# Autodesk Inventor assembly: Assembly1
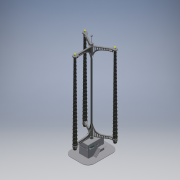
[picture p0: Inventor's stored thumbnail of the model, 180x180]
Saved by Autodesk Inventor 2018 (Build 220112000, 112)
## iProperties
Created: 2017-12-24
Part Number: Assembly1
Document SubType Name: Assembly
Designer: Hembramone
Author: Hembramone
## Documents named in this file (8)
- D:\New folder\mars rotor\Assembly1.iam
- D:\New folder\mars rotor\base rotor.ipt
- D:\New folder\mars rotor\motor.ipt
- D:\New folder\mars rotor\base.ipt
- D:\New folder\mars rotor\transmission box.ipt
- D:\New folder\mars rotor\generator.ipt
- D:\New folder\mars rotor\lightning protector.ipt
- D:\New folder\mars rotor\base support1.ipt
## Components (9 placed, 7 different names)
1. base rotor:1 — Rotational:2, Rotational:3, Flush:1, Flush:3, Rotational:4, Rigid:1, Rotational:5
2. motor:1 — Rigid:1
3. motor:2 — Rotational:2, Rotational:4
4. motor:3 — Rotational:3
5. base:1 — Flush:1, Flush:5
6. transmission box:1 — Flush:3, Flush:4, Rotational:5, Flush:6
7. generator:1 — Flush:4
8. lightning protector:1 — Flush:5
9. base support1:1 — Flush:6
## Relationships (10: Flush 5, RevoluteJoint 4, WeldJoint 1)
- Rotational:2 [RevoluteJoint]: base rotor:1 ↔ motor:2
- Rotational:3 [RevoluteJoint]: base rotor:1 ↔ motor:3
- Flush:1: base rotor:1 ↔ base:1
- Flush:3: base rotor:1 ↔ transmission box:1
- Flush:4: transmission box:1 ↔ generator:1
- Rotational:4 [RevoluteJoint]: base rotor:1 ↔ motor:2
- Rigid:1 [WeldJoint]: base rotor:1 ↔ motor:1
- Rotational:5 [RevoluteJoint]: base rotor:1 ↔ transmission box:1
- Flush:5: base:1 ↔ lightning protector:1
- Flush:6: transmission box:1 ↔ base support1:1
